# Autodesk Inventor assembly: kneader assembly
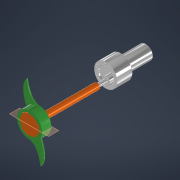
[picture p0: Inventor's stored thumbnail of the model, 180x180]
Saved by Autodesk Inventor 2021 (Build 250183000, 183)
## iProperties
Created: 2022-05-20
Part Number: kneader assembly
Document SubType Name: Assembly
Designer: techv
Author: techv
## Documents named in this file (4)
- D:\Projects\P_Baker Bot\Design\kneader assembly.iam
- D:\Projects\P_Baker Bot\Design\kneading shaft.ipt
- D:\Projects\P_Baker Bot\Design\kneading blade.ipt
- C:\Users\techv\Downloads\JHONSON 12V DC GEARED MOTOR.ipt
## Components (3 placed, 3 different names)
1. kneading shaft:1 — Flush:1, Mate:1, Mate:2
2. kneading blade:1 — Flush:1
3. JHONSON 12V DC GEARED MOTOR:1 — Mate:1, Mate:2
## Relationships (3: Mate 2, Flush 1)
- Flush:1: kneading shaft:1 ↔ kneading blade:1
- Mate:1: kneading shaft:1 ↔ JHONSON 12V DC GEARED MOTOR:1
- Mate:2: kneading shaft:1 ↔ JHONSON 12V DC GEARED MOTOR:1
